# Autodesk Inventor assembly: Odometry module
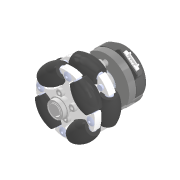
[picture p0: Inventor's stored thumbnail of the model, 180x180]
Saved by Autodesk Inventor 2020 (Build 240168000, 168)
## iProperties
Created: 2019-11-05
Part Number: Odometry module
Document SubType Name: Assembly
Designer: ball
Author: ball
## Documents named in this file (8)
- C:\FTC\FTC8863CAD\2019 Robot\Odoemetry module\Odometry module gb.iam
- C:\FTC\FTC8863CAD\2019 Robot\Odoemetry module\Odometry_Holder.ipt
- C:\FTC\FTC8863CAD\Actobotics\535 parts\535042.ipt
- C:\FTC\FTC8863CAD\Actobotics\634 parts\634064.ipt
- C:\FTC\FTC8863CAD\2019 Robot\Odoemetry module\wheel_dual.iam
- C:\FTC\FTC8863CAD\2019 Robot\Odoemetry module\NewBigSpacer.ipt
- C:\FTC\FTC8863CAD\2019 Robot\Odoemetry module\E8T-X-250-S-D-D-X.iam
- C:\FTC\FTC8863CAD\2019 Robot\Odoemetry module\90576A161_MEDIUM-STRENGTH STEEL NYLON-INSERT LOCKNUT.ipt
## Components (9 placed, 7 different names)
1. Odometry_Holder:1 — Mate:1, Mate:2, Mate:3, Mate:4, Flush:1, Mate:10, Mate:11, Mate:12, Mate:13, Mate:14
2. 535042:1 — Mate:1, Mate:2, Mate:8
3. 535042:2 — Mate:3, Mate:4, Mate:5
4. 634064:1 — Mate:5, Flush:1, Mate:6, Mate:7
5. wheel_dual:1 [sub-assembly] — Mate:6, Mate:17
6. NewBigSpacer:1 — Mate:7, Mate:8, Mate:17
7. E8T-X-250-S-D-D-X:1 [sub-assembly] — Mate:10, Mate:11, Mate:12, Mate:15, Mate:16
8. 90576A161_MEDIUM-STRENGTH STEEL NYLON-INSERT LOCKNUT:1 — Mate:13, Mate:16
9. 90576A161_MEDIUM-STRENGTH STEEL NYLON-INSERT LOCKNUT:2 — Mate:14, Mate:15
## Relationships (17: Mate 16, Flush 1)
- Mate:1: Odometry_Holder:1 ↔ 535042:1
- Mate:2: Odometry_Holder:1 ↔ 535042:1
- Mate:3: Odometry_Holder:1 ↔ 535042:2
- Mate:4: Odometry_Holder:1 ↔ 535042:2
- Mate:5: 535042:2 ↔ 634064:1
- Flush:1: Odometry_Holder:1 ↔ 634064:1
- Mate:6: 634064:1 ↔ wheel_dual:1
- Mate:7: 634064:1 ↔ NewBigSpacer:1
- Mate:8: 535042:1 ↔ NewBigSpacer:1
- Mate:10: Odometry_Holder:1 ↔ E8T-X-250-S-D-D-X:1
- Mate:11: Odometry_Holder:1 ↔ E8T-X-250-S-D-D-X:1
- Mate:12: Odometry_Holder:1 ↔ E8T-X-250-S-D-D-X:1
- Mate:13: Odometry_Holder:1 ↔ 90576A161_MEDIUM-STRENGTH STEEL NYLON-INSERT LOCKNUT:1
- Mate:14: Odometry_Holder:1 ↔ 90576A161_MEDIUM-STRENGTH STEEL NYLON-INSERT LOCKNUT:2
- Mate:15: E8T-X-250-S-D-D-X:1 ↔ 90576A161_MEDIUM-STRENGTH STEEL NYLON-INSERT LOCKNUT:2
- Mate:16: E8T-X-250-S-D-D-X:1 ↔ 90576A161_MEDIUM-STRENGTH STEEL NYLON-INSERT LOCKNUT:1
- Mate:17: wheel_dual:1 ↔ NewBigSpacer:1
